# Autodesk Inventor assembly: Servo Block
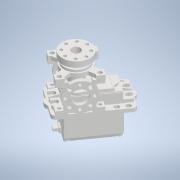
[picture p0: Inventor's stored thumbnail of the model, 180x180]
Saved by Autodesk Inventor 2020 (Build 240168000, 168)
## iProperties
Created: 2020-01-18
Part Number: Servo Block
Document SubType Name: Assembly
Designer: kevin.nguyen
Author: kevin.nguyen
## Documents named in this file (6)
- C:\Users\tdmp4\OneDrive\Documents\GitHub\CAD-2020\ServoCity\Servo Block.iam
- C:\Users\tdmp4\OneDrive\Documents\GitHub\CAD-2020\ServoCity\535118 assembly.iam
- C:\Users\tdmp4\OneDrive\Documents\GitHub\CAD-2020\ServoCity\525123.ipt
- C:\Users\tdmp4\OneDrive\Documents\GitHub\CAD-2020\ServoCity\545420.ipt
- C:\Users\tdmp4\OneDrive\Documents\GitHub\CAD-2020\ServoCity\575112.ipt
- C:\Users\tdmp4\OneDrive\Documents\GitHub\CAD-2020\ServoCity\2000-0025-0002.ipt
## Components (6 placed, 5 different names)
1. 535118 assembly:1 [sub-assembly] — Mate:5, Mate:7, Mate:8, Insert:1, Mate:12, Mate:18, Mate:19
2. 525123:1 — Insert:1
3. 545420:1 — Mate:7, Mate:12, Mate:17, Flush:1, Flush:2, Mate:18, Mate:19
4. 545420:2 — Mate:5, Mate:8
5. 575112:1 — Mate:13, Mate:14, Mate:15, Mate:17, Flush:1, Flush:2
6. 2000-0025-0002:1 — Mate:13, Mate:14, Mate:15
## Relationships (13: Mate 10, Flush 2, Insert 1)
- Mate:5: 535118 assembly:1 ↔ 545420:2
- Mate:7: 535118 assembly:1 ↔ 545420:1
- Mate:8: 535118 assembly:1 ↔ 545420:2
- Insert:1 (3.048 mm): 535118 assembly:1 ↔ 525123:1
- Mate:12: 535118 assembly:1 ↔ 545420:1
- Mate:13: 575112:1 ↔ 2000-0025-0002:1
- Mate:14: 575112:1 ↔ 2000-0025-0002:1
- Mate:15: 575112:1 ↔ 2000-0025-0002:1
- Mate:17: 545420:1 ↔ 575112:1
- Flush:1: 545420:1 ↔ 575112:1
- Flush:2 (2.54 mm): 545420:1 ↔ 575112:1
- Mate:18: 535118 assembly:1 ↔ 545420:1
- Mate:19: 535118 assembly:1 ↔ 545420:1
